# Autodesk Inventor assembly: 肩_1
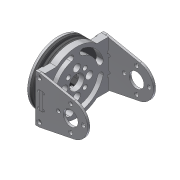
[picture p0: Inventor's stored thumbnail of the model, 180x180]
Saved by Autodesk Inventor 2016 (Build 200138000, 138)
## iProperties
Created: 2016-05-05
Part Number: 肩_1
Document SubType Name: Assembly
Designer: hiroaki
Mass: 31.2319 g
Surface Area: 187.261 cm^2
Volume: 14.2636 cm^3
Density: 2.18962 g/cm^3
Author: hiroaki
## Documents named in this file (7)
- C:\Users\hiro\Documents\kenkyuu\二足\二足ver6.0\上半身\腕\肩_1.iam
- C:\Users\hiro\Documents\kenkyuu\二足\二足ver6.0\上半身\腕\肩_メインフレーム_1_1.ipt
- C:\Users\hiro\Documents\kenkyuu\二足\二足ver6.0\上半身\腕\肩_サブフレーム_1_1.ipt
- C:\Users\hiro\Documents\kenkyuu\二足\二足ver6.0\既製品\BA2542\core_BA2542.ipt
- C:\Users\hiro\Documents\kenkyuu\二足\二足ver6.0\既製品\BA2542\washer_BA2542.ipt
- C:\Users\hiro\Documents\kenkyuu\二足\二足ver6.0\下半身\付け根ロール\付け根ロール_サブフレーム_1_4.ipt
- C:\Users\hiro\Documents\kenkyuu\二足\二足ver6.0\既製品\SLCG5_5-6.ipt
## Components (11 placed, 6 different names)
1. 肩_メインフレーム_1_1:1 — 挿入:1, 挿入:2, 挿入:3, 挿入:4, 挿入:9, 挿入:16, 挿入:17, 挿入:18, 挿入:19
2. 肩_サブフレーム_1_1:1 — 挿入:3, 挿入:4
3. 肩_サブフレーム_1_1:2 — 挿入:1, 挿入:2
4. core_BA2542:1 — 挿入:10
5. washer_BA2542:1 — 挿入:9, 挿入:10
6. core_BA2542:2 — 挿入:15
7. 付け根ロール_サブフレーム_1_4:1 — 挿入:15, 挿入:20, 挿入:21, 挿入:22
8. SLCG5_5-6:1 — 挿入:16, 挿入:21
9. SLCG5_5-6:2 — 挿入:17, 挿入:22
10. SLCG5_5-6:3 — 挿入:18
11. SLCG5_5-6:4 — 挿入:19, 挿入:20
## Relationships (14: Insert 14)
- 挿入:1 [Insert]: 肩_メインフレーム_1_1:1 ↔ 肩_サブフレーム_1_1:2
- 挿入:2 [Insert]: 肩_メインフレーム_1_1:1 ↔ 肩_サブフレーム_1_1:2
- 挿入:3 [Insert]: 肩_メインフレーム_1_1:1 ↔ 肩_サブフレーム_1_1:1
- 挿入:4 [Insert]: 肩_メインフレーム_1_1:1 ↔ 肩_サブフレーム_1_1:1
- 挿入:9 [Insert]: 肩_メインフレーム_1_1:1 ↔ washer_BA2542:1
- 挿入:10 [Insert]: core_BA2542:1 ↔ washer_BA2542:1
- 挿入:15 [Insert]: core_BA2542:2 ↔ 付け根ロール_サブフレーム_1_4:1
- 挿入:16 [Insert]: 肩_メインフレーム_1_1:1 ↔ SLCG5_5-6:1
- 挿入:17 [Insert]: 肩_メインフレーム_1_1:1 ↔ SLCG5_5-6:2
- 挿入:18 [Insert]: 肩_メインフレーム_1_1:1 ↔ SLCG5_5-6:3
- 挿入:19 [Insert]: 肩_メインフレーム_1_1:1 ↔ SLCG5_5-6:4
- 挿入:20 [Insert]: 付け根ロール_サブフレーム_1_4:1 ↔ SLCG5_5-6:4
- 挿入:21 [Insert]: 付け根ロール_サブフレーム_1_4:1 ↔ SLCG5_5-6:1
- 挿入:22 [Insert]: 付け根ロール_サブフレーム_1_4:1 ↔ SLCG5_5-6:2
